# Autodesk Inventor assembly: Aligner Helper Assembly
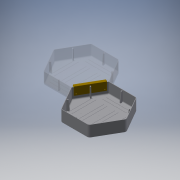
[picture p0: Inventor's stored thumbnail of the model, 180x180]
Saved by Autodesk Inventor 2019 (Build 230136000, 136)
## iProperties
Created: 2021-08-15
Part Number: Aligner Helper Assembly
Document SubType Name: Assembly
Designer: Lix
Author: Lix
## Documents named in this file (3)
- G:\Project\Hybrids\HexaWall\Inventor\Aligner Helper Assembly.iam
- G:\Project\Hybrids\HexaWall\Inventor\Base v6 - 175.ipt
- G:\Project\Hybrids\HexaWall\Inventor\Aligner Helper v2.ipt
## Components (3 placed, 2 different names)
1. Base v6 - 175:1 — Mate:1, Flush:1, Flush:2
2. Base v6 - 175:2 — Mate:1, Flush:1, Flush:2, Mate:2, Mate:3, Mate:4
3. Aligner Helper v2:1 — Mate:2, Mate:3, Mate:4
## Relationships (6: Mate 4, Flush 2)
- Mate:1: Base v6 - 175:1 ↔ Base v6 - 175:2
- Flush:1: Base v6 - 175:1 ↔ Base v6 - 175:2
- Flush:2: Base v6 - 175:1 ↔ Base v6 - 175:2
- Mate:2: Base v6 - 175:2 ↔ Aligner Helper v2:1
- Mate:3: Base v6 - 175:2 ↔ Aligner Helper v2:1
- Mate:4: Base v6 - 175:2 ↔ Aligner Helper v2:1
